# Autodesk Inventor assembly: DraftAssembly
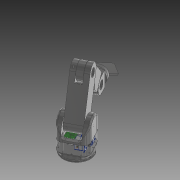
[picture p0: Inventor's stored thumbnail of the model, 180x180]
Saved by Autodesk Inventor 2020 (Build 240168000, 168)
## iProperties
Created: 2021-03-19
Part Number: DraftAssembly
Document SubType Name: Assembly
Designer: DDeGo
Author: DDeGo
## Documents named in this file (34)
- C:\Users\DDeGo\Documents\Drew\Projects\OS-ARM\cad\FirstDraft\DraftAssembly.iam
- C:\Users\DDeGo\Documents\Drew\Projects\OS-ARM\cad\FirstDraft\Base.ipt
- C:\Users\DDeGo\Documents\Drew\Projects\OS-ARM\cad\FirstDraft\Link1.ipt
- C:\Users\DDeGo\Documents\Drew\Projects\OS-ARM\cad\FirstDraft\Link2.ipt
- C:\Users\DDeGo\Documents\Drew\Projects\OS-ARM\cad\FirstDraft\CamBracket.ipt
- C:\Users\DDeGo\Documents\Drew\Projects\OS-ARM\cad\FirstDraft\Wrist.ipt
- C:\Users\DDeGo\Documents\Drew\Projects\OS-ARM\cad\FirstDraft\J1_Base.ipt
- C:\Users\DDeGo\Documents\Drew\Projects\OS-ARM\cad\FirstDraft\Link3.ipt
- C:\Users\DDeGo\Documents\Drew\Projects\OS-ARM\cad\OTS\Electronics\NEMA 23 - 41mm.ipt
- C:\Users\DDeGo\Documents\Drew\Projects\OS-ARM\cad\HarmonicDrive75mm\HarmonicDrive75mm.iam
- C:\Users\DDeGo\Documents\Drew\Projects\OS-ARM\cad\OTS\Radial Bearings\6815 bearing.ipt
- C:\Users\DDeGo\Documents\Drew\Projects\OS-ARM\cad\OTS\Electronics\Nema 17 22mm.ipt
- C:\Users\DDeGo\Documents\Drew\Projects\OS-ARM\cad\FirstDraft\J0_BaseMotorMount.ipt
- C:\Users\DDeGo\Documents\Drew\Projects\OS-ARM\cad\OTS\Radial Bearings\608 bearing.ipt
- C:\Users\DDeGo\Documents\Drew\Projects\OS-ARM\cad\OTS\Thrust Bearings\AXK7095 thrust bearing.ipt
- C:\Users\DDeGo\Documents\Drew\Projects\OS-ARM\cad\FirstDraft\J0_BaseMotorMount2.ipt
- C:\Users\DDeGo\Documents\Drew\Projects\OS-ARM\cad\FirstDraft\J0_DriveDisc.ipt
- C:\Users\DDeGo\Documents\Drew\Projects\OS-ARM\cad\FirstDraft\J1_NewBase.ipt
- C:\Users\DDeGo\Documents\Drew\Projects\OS-ARM\cad\OTS\Electronics\40mmFan.ipt
- C:\Users\DDeGo\Documents\Drew\Projects\OS-ARM\cad\OTS\Radial Bearings\6810 bearing.ipt
- C:\Users\DDeGo\Documents\Drew\Projects\OS-ARM\cad\FirstDraft\J1_NewBaseHDSide.ipt
- C:\Users\DDeGo\Documents\Drew\Projects\OS-ARM\cad\FirstDraft\SmallEncoder.ipt
- C:\Users\DDeGo\Documents\Drew\Projects\OS-ARM\cad\FirstDraft\MotherboardV1\MotherboardV1.ipt
- C:\Users\DDeGo\Documents\Drew\Projects\OS-ARM\cad\FirstDraft\J0_EncoderBracket.ipt
- C:\Users\DDeGo\Documents\Drew\Projects\OS-ARM\cad\FirstDraft\J0_Post.ipt
- C:\Users\DDeGo\Documents\Drew\Projects\OS-ARM\cad\OTS\Other\DiametricMagnet 1-4 x 1-8.ipt
- C:\Users\DDeGo\Documents\Drew\Projects\OS-ARM\cad\FirstDraft\DraftAssembly\Design Accelerator\Spur Gears1.iam
- C:\Users\DDeGo\Documents\Drew\Projects\OS-ARM\cad\FirstDraft\J0_DriveGear.ipt
- C:\Users\DDeGo\Documents\Drew\Projects\OS-ARM\cad\OTS\Radial Bearings\688 bearing.ipt
- C:\Users\DDeGo\Documents\Drew\Projects\OS-ARM\cad\FirstDraft\J1_EncoderGear.ipt
- C:\Users\DDeGo\Documents\Drew\Projects\OS-ARM\cad\FirstDraft\DraftAssembly\Design Accelerator\Spur Gears2.iam
- C:\Users\DDeGo\Documents\Drew\Projects\OS-ARM\cad\OTS\Other\M8x160mm Threaded Rod.ipt
- C:\Users\DDeGo\Documents\Drew\Projects\OS-ARM\cad\OTS\Other\GT2 20T Drive Pulley.ipt
- C:\Users\DDeGo\Documents\Drew\Projects\OS-ARM\cad\FirstDraft\J1_DrivenPulley.ipt
## Components (46 placed, 33 different names)
1. Base:1 — Mate:57, Mate:87, Flush:11, Flush:12, Flush:13, Mate:106, Mate:107, Angle:1, Mate:123
2. Link1:1 — Mate:30, Mate:33, Mate:34, Mate:35, Mate:49, Mate:93, Mate:94, Mate:95, Mate:141, Mate:142, Angle:4, Mate:143, Mate:144, Mate:145, Mate:146, Mate:152, Mate:153, Mate:154, Mate:155
3. Link2:1 — Mate:23, Mate:24, Mate:36, Mate:37, Mate:38, Flush:5, Flush:6, Flush:7, Flush:8, Flush:9, Flush:10
4. CamBracket:1 — Mate:9, Mate:12
5. Wrist:1 — Mate:9, Mate:12, Mate:25, Mate:26
6. J1_Base:1 — Mate:80, Mate:81, Mate:82, Mate:92, Mate:96, Mate:97, Mate:98, Mate:99, Mate:113, Mate:162, Mate:163, Mate:164, Mate:174, Mate:175, Mate:176
7. Link3:1 — Mate:23, Mate:24, Mate:25, Mate:26, Angle:1
8. NEMA 23 - 41mm:1 — Mate:30, Mate:49
9. HarmonicDrive75mm:1 [sub-assembly] — Mate:31, Mate:32, Mate:35, Mate:36, Mate:37, Mate:38
10. 6815 bearing:1 — Mate:31, Mate:32, Mate:33, Mate:34
11. NEMA 23 - 41mm:2 — Mate:169, Mate:174, Mate:175, Mate:176
12. NEMA 23 - 41mm:3 — Mate:77, Mate:78, Mate:79, Mate:138
13. Nema 17 22mm:1 — Flush:5, Flush:6, Flush:7
14. Nema 17 22mm:2 — Flush:8, Flush:9, Flush:10
15. J0_BaseMotorMount:1 — Mate:57, Mate:66, Mate:67, Mate:73, Mate:74, Mate:98, Mate:99, Mate:173
16. 608 bearing:1 — Mate:104, Mate:132, Mate:133
17. AXK7095 thrust bearing:1 — Mate:66, Mate:67, Mate:140
18. J0_BaseMotorMount2:1 — Mate:73, Mate:74, Mate:77, Mate:78, Mate:79, Mate:80, Mate:81, Mate:82, Mate:104, Mate:124, Mate:125, Mate:126, Mate:132, Mate:165, Mate:166, Mate:167
19. J0_DriveDisc:1 — Mate:87, Mate:108, Angle:3, Mate:134, Flush:15, Mate:139, Mate:140, Rotation:1
20. J1_NewBase:1 — Mate:92, Mate:96, Mate:97, Mate:114, Mate:115, Rotation:2, Mate:156, Mate:157, Mate:158, Mate:159, Mate:161
21. 6815 bearing:3 — Mate:88, Mate:90, Mate:111, Mate:112
22. HarmonicDrive75mm:2 [sub-assembly] — Mate:88, Mate:90, Mate:93, Mate:94, Mate:95, Mate:172, Angle:5
23. 40mmFan:1 — Mate:165, Mate:166, Mate:167
24. 6810 bearing:1 — Mate:106, Mate:108, Mate:139
25. AXK7095 thrust bearing:2 — Mate:107, Mate:123, Mate:173
26. J1_NewBaseHDSide:1 — Mate:111, Mate:112, Mate:113, Mate:114, Mate:115, Mate:172
27. SmallEncoder:1 — Mate:127, Mate:128, Angle:2
28. SmallEncoder:2 — Mate:141, Mate:142, Angle:4
29. MotherboardV1:1 — Mate:162, Mate:163, Mate:164
30. J0_EncoderBracket:1 — Mate:124, Mate:125, Mate:126, Mate:127, Mate:128, Angle:2
31. J0_Post:1 — Mate:133, Angle:3, Mate:134, Mate:135, Mate:136
32. DiametricMagnet 1-4 x 1-8:1 — Mate:135, Mate:136
33. J0_DriveGear:1 — Mate:138, Flush:15, Rotation:1
34. J0 Drive Gears [sub-assembly]
35. 688 bearing:1 — Mate:143, Mate:146
36. 688 bearing:2 — Mate:144, Mate:145, Mate:147, Mate:149
37. J1_EncoderGear:1 — Mate:147, Mate:149, Rotation:2, Mate:150, Mate:151
38. J1 Encoder Gears [sub-assembly]
39. DiametricMagnet 1-4 x 1-8:2 — Mate:150, Mate:151
40. 608 bearing:2 — Mate:152, Mate:153, Mate:160
41. 608 bearing:3 — Mate:154, Mate:155
42. 608 bearing:4 — Mate:157, Mate:158, Mate:171
43. 608 bearing:5 — Mate:156, Mate:159
44. M8x160mm Threaded Rod:1 — Mate:160, Mate:161, Mate:170
45. GT2 20T Drive Pulley:1 — Mate:169, Flush:16, Rotation:3
46. J1_DrivenPulley:1 — Mate:170, Mate:171, Flush:16, Rotation:3, Angle:5
## Relationships (114: Mate 95, Flush 11, Angle 5, RelateRotation 3)
- Mate:9: CamBracket:1 ↔ Wrist:1
- Mate:12: CamBracket:1 ↔ Wrist:1
- Mate:23: Link2:1 ↔ Link3:1
- Mate:24: Link2:1 ↔ Link3:1
- Mate:25: Wrist:1 ↔ Link3:1
- Mate:26: Wrist:1 ↔ Link3:1
- Mate:30 (5 mm): Link1:1 ↔ NEMA 23 - 41mm:1
- Mate:31: HarmonicDrive75mm:1 ↔ 6815 bearing:1
- Mate:32: HarmonicDrive75mm:1 ↔ 6815 bearing:1
- Mate:33: Link1:1 ↔ 6815 bearing:1
- Mate:34: Link1:1 ↔ 6815 bearing:1
- Mate:35: Link1:1 ↔ HarmonicDrive75mm:1
- Mate:36: Link2:1 ↔ HarmonicDrive75mm:1
- Mate:37: Link2:1 ↔ HarmonicDrive75mm:1
- Mate:38: Link2:1 ↔ HarmonicDrive75mm:1
- Mate:49: Link1:1 ↔ NEMA 23 - 41mm:1
- Flush:5 (-25 mm): Link2:1 ↔ Nema 17 22mm:1
- Flush:6 (-3 mm): Link2:1 ↔ Nema 17 22mm:1
- Flush:7 (100 mm): Link2:1 ↔ Nema 17 22mm:1
- Flush:8 (-45 mm): Link2:1 ↔ Nema 17 22mm:2
- Flush:9 (55 mm): Link2:1 ↔ Nema 17 22mm:2
- Flush:10 (-25 mm): Link2:1 ↔ Nema 17 22mm:2
- Mate:57: Base:1 ↔ J0_BaseMotorMount:1
- Mate:66: J0_BaseMotorMount:1 ↔ AXK7095 thrust bearing:1
- Mate:67: J0_BaseMotorMount:1 ↔ AXK7095 thrust bearing:1
- Mate:73: J0_BaseMotorMount:1 ↔ J0_BaseMotorMount2:1
- Mate:74: J0_BaseMotorMount:1 ↔ J0_BaseMotorMount2:1
- Mate:77: NEMA 23 - 41mm:3 ↔ J0_BaseMotorMount2:1
- Mate:78: NEMA 23 - 41mm:3 ↔ J0_BaseMotorMount2:1
- Mate:79: NEMA 23 - 41mm:3 ↔ J0_BaseMotorMount2:1
- Mate:80: J1_Base:1 ↔ J0_BaseMotorMount2:1
- Mate:81: J1_Base:1 ↔ J0_BaseMotorMount2:1
- Mate:82: J1_Base:1 ↔ J0_BaseMotorMount2:1
- Mate:87: Base:1 ↔ J0_DriveDisc:1
- Mate:88: 6815 bearing:3 ↔ HarmonicDrive75mm:2
- Mate:90: 6815 bearing:3 ↔ HarmonicDrive75mm:2
- Mate:92: J1_Base:1 ↔ J1_NewBase:1
- Mate:93: Link1:1 ↔ HarmonicDrive75mm:2
- Mate:94: Link1:1 ↔ HarmonicDrive75mm:2
- Mate:95: Link1:1 ↔ HarmonicDrive75mm:2
- Mate:96: J1_Base:1 ↔ J1_NewBase:1
- Mate:97: J1_Base:1 ↔ J1_NewBase:1
- Mate:98: J1_Base:1 ↔ J0_BaseMotorMount:1
- Mate:99: J1_Base:1 ↔ J0_BaseMotorMount:1
- Flush:11: Base:1
- Flush:12: Base:1
- Flush:13: Base:1
- Mate:104: 608 bearing:1 ↔ J0_BaseMotorMount2:1
- Mate:106: Base:1 ↔ 6810 bearing:1
- Mate:107: Base:1 ↔ AXK7095 thrust bearing:2
- Mate:108: J0_DriveDisc:1 ↔ 6810 bearing:1
- Angle:1 (0 deg): Base:1 ↔ Link3:1
- Mate:111: 6815 bearing:3 ↔ J1_NewBaseHDSide:1
- Mate:112: 6815 bearing:3 ↔ J1_NewBaseHDSide:1
- Mate:113: J1_Base:1 ↔ J1_NewBaseHDSide:1
- Mate:114: J1_NewBase:1 ↔ J1_NewBaseHDSide:1
- Mate:115: J1_NewBase:1 ↔ J1_NewBaseHDSide:1
- Mate:123: Base:1 ↔ AXK7095 thrust bearing:2
- Mate:124: J0_BaseMotorMount2:1 ↔ J0_EncoderBracket:1
- Mate:125: J0_BaseMotorMount2:1 ↔ J0_EncoderBracket:1
- Mate:126: J0_BaseMotorMount2:1 ↔ J0_EncoderBracket:1
- Mate:127: SmallEncoder:1 ↔ J0_EncoderBracket:1
- Mate:128: SmallEncoder:1 ↔ J0_EncoderBracket:1
- Angle:2 (0 deg): SmallEncoder:1 ↔ J0_EncoderBracket:1
- Mate:132: 608 bearing:1 ↔ J0_BaseMotorMount2:1
- Mate:133: 608 bearing:1 ↔ J0_Post:1
- Angle:3 (0 deg): J0_DriveDisc:1 ↔ J0_Post:1
- Mate:134: J0_DriveDisc:1 ↔ J0_Post:1
- Mate:135: J0_Post:1 ↔ DiametricMagnet 1-4 x 1-8:1
- Mate:136: J0_Post:1 ↔ DiametricMagnet 1-4 x 1-8:1
- Mate:138: NEMA 23 - 41mm:3 ↔ J0_DriveGear:1
- Flush:15: J0_DriveDisc:1 ↔ J0_DriveGear:1
- Mate:139: J0_DriveDisc:1 ↔ 6810 bearing:1
- Mate:140: AXK7095 thrust bearing:1 ↔ J0_DriveDisc:1
- Rotation:1 [RelateRotation] (0.13 ul): J0_DriveDisc:1 ↔ J0_DriveGear:1
- Mate:141: Link1:1 ↔ SmallEncoder:2
- Mate:142: Link1:1 ↔ SmallEncoder:2
- Angle:4 (0 deg): Link1:1 ↔ SmallEncoder:2
- Mate:143: Link1:1 ↔ 688 bearing:1
- Mate:144: Link1:1 ↔ 688 bearing:2
- Mate:145: Link1:1 ↔ 688 bearing:2
- Mate:146: Link1:1 ↔ 688 bearing:1
- Mate:147: 688 bearing:2 ↔ J1_EncoderGear:1
- Mate:149: 688 bearing:2 ↔ J1_EncoderGear:1
- Rotation:2 [RelateRotation] (0.6667 ul): J1_NewBase:1 ↔ J1_EncoderGear:1
- Mate:150: J1_EncoderGear:1 ↔ DiametricMagnet 1-4 x 1-8:2
- Mate:151: J1_EncoderGear:1 ↔ DiametricMagnet 1-4 x 1-8:2
- Mate:152: Link1:1 ↔ 608 bearing:2
- Mate:153: Link1:1 ↔ 608 bearing:2
- Mate:154: Link1:1 ↔ 608 bearing:3
- Mate:155: Link1:1 ↔ 608 bearing:3
- Mate:156: J1_NewBase:1 ↔ 608 bearing:5
- Mate:157: J1_NewBase:1 ↔ 608 bearing:4
- Mate:158: J1_NewBase:1 ↔ 608 bearing:4
- Mate:159: J1_NewBase:1 ↔ 608 bearing:5
- Mate:160: 608 bearing:2 ↔ M8x160mm Threaded Rod:1
- Mate:161 (1.5 mm): J1_NewBase:1 ↔ M8x160mm Threaded Rod:1
- Mate:162: J1_Base:1 ↔ MotherboardV1:1
- Mate:163: J1_Base:1 ↔ MotherboardV1:1
- Mate:164: J1_Base:1 ↔ MotherboardV1:1
- Mate:165: J0_BaseMotorMount2:1 ↔ 40mmFan:1
- Mate:166: J0_BaseMotorMount2:1 ↔ 40mmFan:1
- Mate:167: J0_BaseMotorMount2:1 ↔ 40mmFan:1
- Mate:169: NEMA 23 - 41mm:2 ↔ GT2 20T Drive Pulley:1
- Mate:170: M8x160mm Threaded Rod:1 ↔ J1_DrivenPulley:1
- Mate:171 (1 mm): 608 bearing:4 ↔ J1_DrivenPulley:1
- Mate:172: HarmonicDrive75mm:2 ↔ J1_NewBaseHDSide:1
- Flush:16: GT2 20T Drive Pulley:1 ↔ J1_DrivenPulley:1
- Rotation:3 [RelateRotation] (3 ul): GT2 20T Drive Pulley:1 ↔ J1_DrivenPulley:1
- Angle:5 (0 deg): HarmonicDrive75mm:2 ↔ J1_DrivenPulley:1
- Mate:173: J0_BaseMotorMount:1 ↔ AXK7095 thrust bearing:2
- Mate:174: J1_Base:1 ↔ NEMA 23 - 41mm:2
- Mate:175: J1_Base:1 ↔ NEMA 23 - 41mm:2
- Mate:176: J1_Base:1 ↔ NEMA 23 - 41mm:2
